# Autodesk Inventor assembly: funnel_mirrored_mirrored
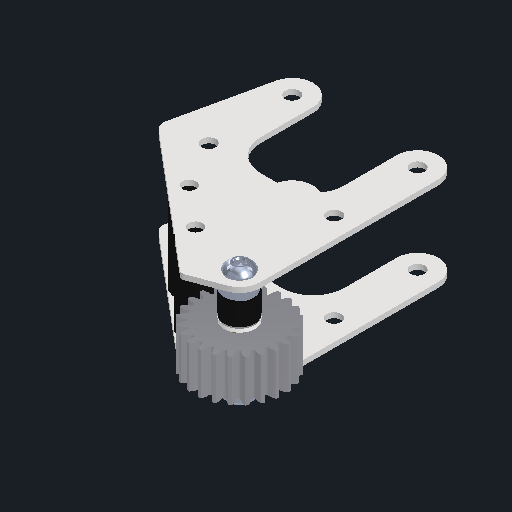
[picture p0: Inventor's stored thumbnail of the model, 512x512]
Saved by Autodesk Inventor 2025 (Build 290162000, 162)
## iProperties
Created: 2024-10-12
Part Number: funnel_mirrored_mirrored
Document SubType Name: Assembly
Designer: Averey Ku
Author: Averey Ku
## Documents named in this file (14)
- D:\vex_robotics_high_stakes\hardware\cad\bots\high_stakes_v2\chassis_v2\drivebay_mirrored\funnel_mirrored_mirrored.iam
- D:\vex_robotics_high_stakes\hardware\cad\bots\high_stakes_v2\chassis_v2\drivebay_mirrored\funel_gusset_mirrored_mirrored.ipt
- D:\vex_robotics_high_stakes\hardware\cad\bots\high_stakes_v2\chassis_v2\drivebay_mirrored\HS 24T Gear, Circle_mirrored_mirrored.iam
- D:\vex_robotics_high_stakes\hardware\cad\robpros_cad_lib\Motion\Spacers\Spacer Nylon .375 OD\NSpacer .375 OD x .500.ipt
- D:\vex_robotics_high_stakes\hardware\cad\robpros_cad_lib\Motion\Spacers\Spacer Nylon .375 OD.ipt
- D:\vex_robotics_high_stakes\hardware\cad\robpros_cad_lib\Motion\Spacers\Washer Teflon\TWasher .375 OD x .04000.ipt
- D:\vex_robotics_high_stakes\hardware\cad\robpros_cad_lib\Motion\Spacers\Washer Teflon.ipt
- D:\vex_robotics_high_stakes\hardware\cad\bots\high_stakes_v2\chassis_v2\drivebay_mirrored\Nut Keps_mirrored_mirrored.ipt
- D:\vex_robotics_high_stakes\hardware\cad\bots\high_stakes_v2\chassis_v2\drivebay_mirrored\Nut Thin Nylock_mirrored_mirrored.ipt
- D:\vex_robotics_high_stakes\hardware\cad\robpros_cad_lib\Motion\Spacers\Spacer Nylon .375 OD\NSpacer .375 OD x .250.ipt
- D:\vex_robotics_high_stakes\hardware\cad\robpros_cad_lib\Motion\Spacers\Washer Steel\SWasher .375 OD x .015625.ipt
- D:\vex_robotics_high_stakes\hardware\cad\robpros_cad_lib\Motion\Spacers\Washer Steel.ipt
- D:\vex_robotics_high_stakes\hardware\cad\robpros_cad_lib\Structure\Hardware\Screw Steel - Star\SScrew Star Smooth 1.250.ipt
- D:\vex_robotics_high_stakes\hardware\cad\robpros_cad_lib\Structure\Hardware\Screw Steel - Star.ipt
## Components (14 placed, 9 different names)
1. funel_gusset_mirrored_mirrored:1 — Insert:3, Insert:5, Insert:10, Insert:15
2. HS 24T Gear, Circle_mirrored_mirrored:1 [sub-assembly] — Insert:8
3. funel_gusset_mirrored_mirrored:2 — Mate:2, Insert:6, Mate:1, Insert:9, Insert:11
4. NSpacer .375 OD x .500:1 — Insert:6, Insert:2
5. NSpacer .375 OD x .500:2 — Insert:2, Insert:3
6. NSpacer .375 OD x .500:3 — Mate:1, Insert:4
7. NSpacer .375 OD x .500:4 — Insert:4, Insert:5
8. TWasher .375 OD x .04000:1 — Insert:8, Insert:9
9. Nut Keps_mirrored_mirrored:1 — Insert:10, Insert:14
10. Nut Thin Nylock_mirrored_mirrored:1 — Insert:11
11. NSpacer .375 OD x .250:5 — Insert:14, Insert:12
12. TWasher .375 OD x .04000:2 — Insert:13
13. SWasher .375 OD x .015625:1 — Insert:12, Insert:13
14. SScrew Star Smooth 1.250:1 — Insert:15
## Relationships (15: Insert 13, Mate 2)
- Mate:2: funel_gusset_mirrored_mirrored:2
- Insert:6: funel_gusset_mirrored_mirrored:2 ↔ NSpacer .375 OD x .500:1
- Insert:2: NSpacer .375 OD x .500:1 ↔ NSpacer .375 OD x .500:2
- Insert:3: funel_gusset_mirrored_mirrored:1 ↔ NSpacer .375 OD x .500:2
- Mate:1: funel_gusset_mirrored_mirrored:2 ↔ NSpacer .375 OD x .500:3
- Insert:4: NSpacer .375 OD x .500:3 ↔ NSpacer .375 OD x .500:4
- Insert:5: funel_gusset_mirrored_mirrored:1 ↔ NSpacer .375 OD x .500:4
- Insert:8: HS 24T Gear, Circle_mirrored_mirrored:1 ↔ TWasher .375 OD x .04000:1
- Insert:9: funel_gusset_mirrored_mirrored:2 ↔ TWasher .375 OD x .04000:1
- Insert:10: funel_gusset_mirrored_mirrored:1 ↔ Nut Keps_mirrored_mirrored:1
- Insert:11: funel_gusset_mirrored_mirrored:2 ↔ Nut Thin Nylock_mirrored_mirrored:1
- Insert:14: Nut Keps_mirrored_mirrored:1 ↔ NSpacer .375 OD x .250:5
- Insert:12: NSpacer .375 OD x .250:5 ↔ SWasher .375 OD x .015625:1
- Insert:13: TWasher .375 OD x .04000:2 ↔ SWasher .375 OD x .015625:1
- Insert:15: funel_gusset_mirrored_mirrored:1 ↔ SScrew Star Smooth 1.250:1
